# Autodesk Inventor assembly: Arrm
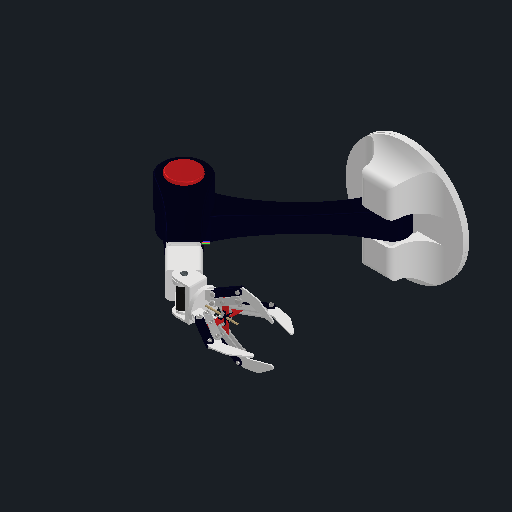
[picture p0: Inventor's stored thumbnail of the model, 512x512]
Saved by Autodesk Inventor 2023 (Build 270158000, 158)
## iProperties
Created: 2023-04-09
Part Number: Arrm
Document SubType Name: Assembly
Designer: vatdu
Author: vatdu
## Documents named in this file (5)
- C:\Users\vatdu\Desktop\CRYSTAL MARK II\Arm\Arm.iam
- C:\Users\vatdu\Desktop\CRYSTAL MARK II\Arm\Shoulder\Shoulder V2.iam
- C:\Users\vatdu\Desktop\CRYSTAL MARK II\Arm\Elbow\Elbow.iam
- C:\Users\vatdu\Desktop\CRYSTAL MARK II\Arm\Wrist\Wrist.iam
- C:\Users\vatdu\Desktop\CRYSTAL MARK II\Arm\Claw\Claw.iam
## Components (4 placed, 4 different names)
1. Shoulder V2:1 [sub-assembly] — Rotational:1
2. Elbow:1 [sub-assembly] — Rotational:1, Rotational:2, Rotational:3
3. Wrist:1 [sub-assembly] — Rotational:2, Rotational:3, Rotational:4
4. Claw:1 [sub-assembly] — Rotational:4
## Relationships (4: RevoluteJoint 4)
- Rotational:1 [RevoluteJoint]: Shoulder V2:1 ↔ Elbow:1
- Rotational:2 [RevoluteJoint] (10 mm): Elbow:1 ↔ Wrist:1
- Rotational:3 [RevoluteJoint] (10 mm): Elbow:1 ↔ Wrist:1
- Rotational:4 [RevoluteJoint]: Wrist:1 ↔ Claw:1
